(part 1 of 2)
# Autodesk Inventor assembly: FRC Fixed Field 2018_sldasm
Saved by Autodesk Inventor 2016 SP2 (Build 200236200, 236)
## iProperties
Created: 2018-01-13
Part Number: FRC Fixed Field 2018_sldasm
Document SubType Name: Assembly
Designer: CAD
Author: CAD
## Documents named in this file (943)
- C:\Users\CAD\Documents\GitHub\FIRST Power Up Field CAD\FRC Fixed Field 2018_sldasm.iam
- C:\Users\CAD\Documents\GitHub\FIRST Power Up Field CAD\Body_525_sldprt.ipt
- C:\Users\CAD\Documents\GitHub\FIRST Power Up Field CAD\Body_526_sldprt.ipt
- C:\Users\CAD\Documents\GitHub\FIRST Power Up Field CAD\Body_527_sldprt.ipt
- C:\Users\CAD\Documents\GitHub\FIRST Power Up Field CAD\Body_528_sldprt.ipt
- C:\Users\CAD\Documents\GitHub\FIRST Power Up Field CAD\Body_529_sldprt.ipt
- C:\Users\CAD\Documents\GitHub\FIRST Power Up Field CAD\Body_530_sldprt.ipt
- C:\Users\CAD\Documents\GitHub\FIRST Power Up Field CAD\Body_531_sldprt.ipt
- C:\Users\CAD\Documents\GitHub\FIRST Power Up Field CAD\Body_532_sldprt.ipt
- C:\Users\CAD\Documents\GitHub\FIRST Power Up Field CAD\Body_533_sldprt.ipt
- C:\Users\CAD\Documents\GitHub\FIRST Power Up Field CAD\Body_534_sldprt.ipt
- C:\Users\CAD\Documents\GitHub\FIRST Power Up Field CAD\Body_535_sldprt.ipt
- C:\Users\CAD\Documents\GitHub\FIRST Power Up Field CAD\Body_536_sldprt.ipt
- C:\Users\CAD\Documents\GitHub\FIRST Power Up Field CAD\Body_537_sldprt.ipt
- C:\Users\CAD\Documents\GitHub\FIRST Power Up Field CAD\Body_538_sldprt.ipt
- C:\Users\CAD\Documents\GitHub\FIRST Power Up Field CAD\Body_539_sldprt.ipt
- C:\Users\CAD\Documents\GitHub\FIRST Power Up Field CAD\Body_540_sldprt.ipt
- C:\Users\CAD\Documents\GitHub\FIRST Power Up Field CAD\Body_541_sldprt.ipt
- C:\Users\CAD\Documents\GitHub\FIRST Power Up Field CAD\Body_542_sldprt.ipt
- C:\Users\CAD\Documents\GitHub\FIRST Power Up Field CAD\Body_543_sldprt.ipt
- C:\Users\CAD\Documents\GitHub\FIRST Power Up Field CAD\Body_544_sldprt.ipt
- C:\Users\CAD\Documents\GitHub\FIRST Power Up Field CAD\Body_545_sldprt.ipt
- C:\Users\CAD\Documents\GitHub\FIRST Power Up Field CAD\Body_546_sldprt.ipt
- C:\Users\CAD\Documents\GitHub\FIRST Power Up Field CAD\Body_547_sldprt.ipt
- C:\Users\CAD\Documents\GitHub\FIRST Power Up Field CAD\Body_548_sldprt.ipt
- C:\Users\CAD\Documents\GitHub\FIRST Power Up Field CAD\Body_549_sldprt.ipt
- C:\Users\CAD\Documents\GitHub\FIRST Power Up Field CAD\Body_550_sldprt.ipt
- C:\Users\CAD\Documents\GitHub\FIRST Power Up Field CAD\Body_551_sldprt.ipt
- C:\Users\CAD\Documents\GitHub\FIRST Power Up Field CAD\Body_552_sldprt.ipt
- C:\Users\CAD\Documents\GitHub\FIRST Power Up Field CAD\Body_553_sldprt.ipt
- C:\Users\CAD\Documents\GitHub\FIRST Power Up Field CAD\Body_554_sldprt.ipt
- C:\Users\CAD\Documents\GitHub\FIRST Power Up Field CAD\Body_555_sldprt.ipt
- C:\Users\CAD\Documents\GitHub\FIRST Power Up Field CAD\Body_556_sldprt.ipt
- C:\Users\CAD\Documents\GitHub\FIRST Power Up Field CAD\Body_557_sldprt.ipt
- C:\Users\CAD\Documents\GitHub\FIRST Power Up Field CAD\Body_558_sldprt.ipt
- C:\Users\CAD\Documents\GitHub\FIRST Power Up Field CAD\Body_559_sldprt.ipt
- C:\Users\CAD\Documents\GitHub\FIRST Power Up Field CAD\Body_560_sldprt.ipt
- C:\Users\CAD\Documents\GitHub\FIRST Power Up Field CAD\Body_561_sldprt.ipt
- C:\Users\CAD\Documents\GitHub\FIRST Power Up Field CAD\Body_562_sldprt.ipt
- C:\Users\CAD\Documents\GitHub\FIRST Power Up Field CAD\Body_563_sldprt.ipt
- C:\Users\CAD\Documents\GitHub\FIRST Power Up Field CAD\Body_564_sldprt.ipt
- C:\Users\CAD\Documents\GitHub\FIRST Power Up Field CAD\Body_565_sldprt.ipt
- C:\Users\CAD\Documents\GitHub\FIRST Power Up Field CAD\Body_566_sldprt.ipt
- C:\Users\CAD\Documents\GitHub\FIRST Power Up Field CAD\Body_567_sldprt.ipt
- C:\Users\CAD\Documents\GitHub\FIRST Power Up Field CAD\Body_568_sldprt.ipt
- C:\Users\CAD\Documents\GitHub\FIRST Power Up Field CAD\Body_569_sldprt.ipt
- C:\Users\CAD\Documents\GitHub\FIRST Power Up Field CAD\Body_570_sldprt.ipt
- C:\Users\CAD\Documents\GitHub\FIRST Power Up Field CAD\Body_571_sldprt.ipt
- C:\Users\CAD\Documents\GitHub\FIRST Power Up Field CAD\Body_572_sldprt.ipt
- C:\Users\CAD\Documents\GitHub\FIRST Power Up Field CAD\Body_573_sldprt.ipt
- C:\Users\CAD\Documents\GitHub\FIRST Power Up Field CAD\Body_574_sldprt.ipt
- C:\Users\CAD\Documents\GitHub\FIRST Power Up Field CAD\Body_575_sldprt.ipt
- C:\Users\CAD\Documents\GitHub\FIRST Power Up Field CAD\Body_576_sldprt.ipt
- C:\Users\CAD\Documents\GitHub\FIRST Power Up Field CAD\Body_577_sldprt.ipt
- C:\Users\CAD\Documents\GitHub\FIRST Power Up Field CAD\Body_578_sldprt.ipt
- C:\Users\CAD\Documents\GitHub\FIRST Power Up Field CAD\Body_579_sldprt.ipt
- C:\Users\CAD\Documents\GitHub\FIRST Power Up Field CAD\Body_580_sldprt.ipt
- C:\Users\CAD\Documents\GitHub\FIRST Power Up Field CAD\Body_581_sldprt.ipt
- C:\Users\CAD\Documents\GitHub\FIRST Power Up Field CAD\Body_582_sldprt.ipt
- C:\Users\CAD\Documents\GitHub\FIRST Power Up Field CAD\Body_583_sldprt.ipt
- C:\Users\CAD\Documents\GitHub\FIRST Power Up Field CAD\Body_584_sldprt.ipt
- C:\Users\CAD\Documents\GitHub\FIRST Power Up Field CAD\Body_585_sldprt.ipt
- C:\Users\CAD\Documents\GitHub\FIRST Power Up Field CAD\Body_586_sldprt.ipt
- C:\Users\CAD\Documents\GitHub\FIRST Power Up Field CAD\Body_587_sldprt.ipt
- C:\Users\CAD\Documents\GitHub\FIRST Power Up Field CAD\Body_588_sldprt.ipt
- C:\Users\CAD\Documents\GitHub\FIRST Power Up Field CAD\Body_589_sldprt.ipt
- C:\Users\CAD\Documents\GitHub\FIRST Power Up Field CAD\Body_590_sldprt.ipt
- C:\Users\CAD\Documents\GitHub\FIRST Power Up Field CAD\Body_591_sldprt.ipt
- C:\Users\CAD\Documents\GitHub\FIRST Power Up Field CAD\Body_592_sldprt.ipt
- C:\Users\CAD\Documents\GitHub\FIRST Power Up Field CAD\Body_593_sldprt.ipt
- C:\Users\CAD\Documents\GitHub\FIRST Power Up Field CAD\Body_594_sldprt.ipt
- C:\Users\CAD\Documents\GitHub\FIRST Power Up Field CAD\Body_595_sldprt.ipt
- C:\Users\CAD\Documents\GitHub\FIRST Power Up Field CAD\Body_596_sldprt.ipt
- C:\Users\CAD\Documents\GitHub\FIRST Power Up Field CAD\Body_597_sldprt.ipt
- C:\Users\CAD\Documents\GitHub\FIRST Power Up Field CAD\Body_598_sldprt.ipt
- C:\Users\CAD\Documents\GitHub\FIRST Power Up Field CAD\Body_599_sldprt.ipt
- C:\Users\CAD\Documents\GitHub\FIRST Power Up Field CAD\Body_600_sldprt.ipt
- C:\Users\CAD\Documents\GitHub\FIRST Power Up Field CAD\Body_601_sldprt.ipt
- C:\Users\CAD\Documents\GitHub\FIRST Power Up Field CAD\Body_602_sldprt.ipt
- C:\Users\CAD\Documents\GitHub\FIRST Power Up Field CAD\Body_603_sldprt.ipt
- C:\Users\CAD\Documents\GitHub\FIRST Power Up Field CAD\Body_604_sldprt.ipt
- C:\Users\CAD\Documents\GitHub\FIRST Power Up Field CAD\Body_605_sldprt.ipt
- C:\Users\CAD\Documents\GitHub\FIRST Power Up Field CAD\Body_606_sldprt.ipt
- C:\Users\CAD\Documents\GitHub\FIRST Power Up Field CAD\Body_607_sldprt.ipt
- C:\Users\CAD\Documents\GitHub\FIRST Power Up Field CAD\Body_608_sldprt.ipt
- C:\Users\CAD\Documents\GitHub\FIRST Power Up Field CAD\Body_609_sldprt.ipt
- C:\Users\CAD\Documents\GitHub\FIRST Power Up Field CAD\Body_610_sldprt.ipt
- C:\Users\CAD\Documents\GitHub\FIRST Power Up Field CAD\Body_611_sldprt.ipt
- C:\Users\CAD\Documents\GitHub\FIRST Power Up Field CAD\Body_612_sldprt.ipt
- C:\Users\CAD\Documents\GitHub\FIRST Power Up Field CAD\Body_613_sldprt.ipt
- C:\Users\CAD\Documents\GitHub\FIRST Power Up Field CAD\Body_614_sldprt.ipt
- C:\Users\CAD\Documents\GitHub\FIRST Power Up Field CAD\Body_615_sldprt.ipt
- C:\Users\CAD\Documents\GitHub\FIRST Power Up Field CAD\Body_616_sldprt.ipt
- C:\Users\CAD\Documents\GitHub\FIRST Power Up Field CAD\Body_617_sldprt.ipt
- C:\Users\CAD\Documents\GitHub\FIRST Power Up Field CAD\Body_618_sldprt.ipt
- C:\Users\CAD\Documents\GitHub\FIRST Power Up Field CAD\Body_619_sldprt.ipt
- C:\Users\CAD\Documents\GitHub\FIRST Power Up Field CAD\Body_620_sldprt.ipt
- C:\Users\CAD\Documents\GitHub\FIRST Power Up Field CAD\Body_621_sldprt.ipt
- C:\Users\CAD\Documents\GitHub\FIRST Power Up Field CAD\Body_622_sldprt.ipt
- C:\Users\CAD\Documents\GitHub\FIRST Power Up Field CAD\Body_623_sldprt.ipt
- C:\Users\CAD\Documents\GitHub\FIRST Power Up Field CAD\Body_624_sldprt.ipt
- C:\Users\CAD\Documents\GitHub\FIRST Power Up Field CAD\Body_625_sldprt.ipt
- C:\Users\CAD\Documents\GitHub\FIRST Power Up Field CAD\Body_626_sldprt.ipt
- C:\Users\CAD\Documents\GitHub\FIRST Power Up Field CAD\Body_627_sldprt.ipt
- C:\Users\CAD\Documents\GitHub\FIRST Power Up Field CAD\Body_628_sldprt.ipt
- C:\Users\CAD\Documents\GitHub\FIRST Power Up Field CAD\Body_629_sldprt.ipt
- C:\Users\CAD\Documents\GitHub\FIRST Power Up Field CAD\Body_630_sldprt.ipt
- C:\Users\CAD\Documents\GitHub\FIRST Power Up Field CAD\Body_631_sldprt.ipt
- C:\Users\CAD\Documents\GitHub\FIRST Power Up Field CAD\Body_632_sldprt.ipt
- C:\Users\CAD\Documents\GitHub\FIRST Power Up Field CAD\Body_633_sldprt.ipt
- C:\Users\CAD\Documents\GitHub\FIRST Power Up Field CAD\Body_634_sldprt.ipt
- C:\Users\CAD\Documents\GitHub\FIRST Power Up Field CAD\Body_635_sldprt.ipt
- C:\Users\CAD\Documents\GitHub\FIRST Power Up Field CAD\Body_636_sldprt.ipt
- C:\Users\CAD\Documents\GitHub\FIRST Power Up Field CAD\Body_637_sldprt.ipt
- C:\Users\CAD\Documents\GitHub\FIRST Power Up Field CAD\Body_638_sldprt.ipt
- C:\Users\CAD\Documents\GitHub\FIRST Power Up Field CAD\Body_639_sldprt.ipt
- C:\Users\CAD\Documents\GitHub\FIRST Power Up Field CAD\Body_640_sldprt.ipt
- C:\Users\CAD\Documents\GitHub\FIRST Power Up Field CAD\Body_641_sldprt.ipt
- C:\Users\CAD\Documents\GitHub\FIRST Power Up Field CAD\Body_642_sldprt.ipt
- C:\Users\CAD\Documents\GitHub\FIRST Power Up Field CAD\Body_643_sldprt.ipt
- C:\Users\CAD\Documents\GitHub\FIRST Power Up Field CAD\Body_644_sldprt.ipt
- C:\Users\CAD\Documents\GitHub\FIRST Power Up Field CAD\Body_645_sldprt.ipt
- C:\Users\CAD\Documents\GitHub\FIRST Power Up Field CAD\Body_646_sldprt.ipt
- C:\Users\CAD\Documents\GitHub\FIRST Power Up Field CAD\Body_647_sldprt.ipt
- C:\Users\CAD\Documents\GitHub\FIRST Power Up Field CAD\Body_648_sldprt.ipt
- C:\Users\CAD\Documents\GitHub\FIRST Power Up Field CAD\Body_649_sldprt.ipt
- C:\Users\CAD\Documents\GitHub\FIRST Power Up Field CAD\Body_650_sldprt.ipt
- C:\Users\CAD\Documents\GitHub\FIRST Power Up Field CAD\Body_651_sldprt.ipt
- C:\Users\CAD\Documents\GitHub\FIRST Power Up Field CAD\Body_652_sldprt.ipt
- C:\Users\CAD\Documents\GitHub\FIRST Power Up Field CAD\Body_653_sldprt.ipt
- C:\Users\CAD\Documents\GitHub\FIRST Power Up Field CAD\Body_654_sldprt.ipt
- C:\Users\CAD\Documents\GitHub\FIRST Power Up Field CAD\Body_655_sldprt.ipt
- C:\Users\CAD\Documents\GitHub\FIRST Power Up Field CAD\Body_656_sldprt.ipt
- C:\Users\CAD\Documents\GitHub\FIRST Power Up Field CAD\Body_657_sldprt.ipt
- C:\Users\CAD\Documents\GitHub\FIRST Power Up Field CAD\Body_658_sldprt.ipt
- C:\Users\CAD\Documents\GitHub\FIRST Power Up Field CAD\Body_659_sldprt.ipt
- C:\Users\CAD\Documents\GitHub\FIRST Power Up Field CAD\Body_660_sldprt.ipt
- C:\Users\CAD\Documents\GitHub\FIRST Power Up Field CAD\Body_661_sldprt.ipt
- C:\Users\CAD\Documents\GitHub\FIRST Power Up Field CAD\Body_662_sldprt.ipt
- C:\Users\CAD\Documents\GitHub\FIRST Power Up Field CAD\Body_663_sldprt.ipt
- C:\Users\CAD\Documents\GitHub\FIRST Power Up Field CAD\Body_664_sldprt.ipt
- C:\Users\CAD\Documents\GitHub\FIRST Power Up Field CAD\Body_665_sldprt.ipt
- C:\Users\CAD\Documents\GitHub\FIRST Power Up Field CAD\Body_666_sldprt.ipt
- C:\Users\CAD\Documents\GitHub\FIRST Power Up Field CAD\Body_667_sldprt.ipt
- C:\Users\CAD\Documents\GitHub\FIRST Power Up Field CAD\Body_668_sldprt.ipt
- C:\Users\CAD\Documents\GitHub\FIRST Power Up Field CAD\Body_669_sldprt.ipt
- C:\Users\CAD\Documents\GitHub\FIRST Power Up Field CAD\Body_670_sldprt.ipt
- C:\Users\CAD\Documents\GitHub\FIRST Power Up Field CAD\Body_671_sldprt.ipt
- C:\Users\CAD\Documents\GitHub\FIRST Power Up Field CAD\Body_672_sldprt.ipt
- C:\Users\CAD\Documents\GitHub\FIRST Power Up Field CAD\Body_673_sldprt.ipt
- C:\Users\CAD\Documents\GitHub\FIRST Power Up Field CAD\Body_674_sldprt.ipt
- C:\Users\CAD\Documents\GitHub\FIRST Power Up Field CAD\Body_675_sldprt.ipt
- C:\Users\CAD\Documents\GitHub\FIRST Power Up Field CAD\Body_676_sldprt.ipt
- C:\Users\CAD\Documents\GitHub\FIRST Power Up Field CAD\Body_677_sldprt.ipt
- C:\Users\CAD\Documents\GitHub\FIRST Power Up Field CAD\Body_678_sldprt.ipt
- C:\Users\CAD\Documents\GitHub\FIRST Power Up Field CAD\Body_679_sldprt.ipt
- C:\Users\CAD\Documents\GitHub\FIRST Power Up Field CAD\Body_680_sldprt.ipt
- C:\Users\CAD\Documents\GitHub\FIRST Power Up Field CAD\Body_681_sldprt.ipt
- C:\Users\CAD\Documents\GitHub\FIRST Power Up Field CAD\Body_682_sldprt.ipt
- C:\Users\CAD\Documents\GitHub\FIRST Power Up Field CAD\Body_683_sldprt.ipt
- C:\Users\CAD\Documents\GitHub\FIRST Power Up Field CAD\Body_684_sldprt.ipt
- C:\Users\CAD\Documents\GitHub\FIRST Power Up Field CAD\Body_685_sldprt.ipt
- C:\Users\CAD\Documents\GitHub\FIRST Power Up Field CAD\Body_686_sldprt.ipt
- C:\Users\CAD\Documents\GitHub\FIRST Power Up Field CAD\Body_687_sldprt.ipt
- C:\Users\CAD\Documents\GitHub\FIRST Power Up Field CAD\Body_688_sldprt.ipt
- C:\Users\CAD\Documents\GitHub\FIRST Power Up Field CAD\Body_689_sldprt.ipt
- C:\Users\CAD\Documents\GitHub\FIRST Power Up Field CAD\Body_690_sldprt.ipt
- C:\Users\CAD\Documents\GitHub\FIRST Power Up Field CAD\Body_691_sldprt.ipt
- C:\Users\CAD\Documents\GitHub\FIRST Power Up Field CAD\Body_692_sldprt.ipt
- C:\Users\CAD\Documents\GitHub\FIRST Power Up Field CAD\Body_693_sldprt.ipt
- C:\Users\CAD\Documents\GitHub\FIRST Power Up Field CAD\Body_694_sldprt.ipt
- C:\Users\CAD\Documents\GitHub\FIRST Power Up Field CAD\Body_695_sldprt.ipt
- C:\Users\CAD\Documents\GitHub\FIRST Power Up Field CAD\Body_696_sldprt.ipt
- C:\Users\CAD\Documents\GitHub\FIRST Power Up Field CAD\Body_697_sldprt.ipt
- C:\Users\CAD\Documents\GitHub\FIRST Power Up Field CAD\Body_698_sldprt.ipt
- C:\Users\CAD\Documents\GitHub\FIRST Power Up Field CAD\Body_699_sldprt.ipt
- C:\Users\CAD\Documents\GitHub\FIRST Power Up Field CAD\Body_700_sldprt.ipt
- C:\Users\CAD\Documents\GitHub\FIRST Power Up Field CAD\Body_701_sldprt.ipt
- C:\Users\CAD\Documents\GitHub\FIRST Power Up Field CAD\Body_702_sldprt.ipt
- C:\Users\CAD\Documents\GitHub\FIRST Power Up Field CAD\Body_703_sldprt.ipt
- C:\Users\CAD\Documents\GitHub\FIRST Power Up Field CAD\Body_704_sldprt.ipt
- C:\Users\CAD\Documents\GitHub\FIRST Power Up Field CAD\Body_705_sldprt.ipt
- C:\Users\CAD\Documents\GitHub\FIRST Power Up Field CAD\Body_706_sldprt.ipt
- C:\Users\CAD\Documents\GitHub\FIRST Power Up Field CAD\Body_707_sldprt.ipt
- C:\Users\CAD\Documents\GitHub\FIRST Power Up Field CAD\Body_708_sldprt.ipt
- C:\Users\CAD\Documents\GitHub\FIRST Power Up Field CAD\Body_709_sldprt.ipt
- C:\Users\CAD\Documents\GitHub\FIRST Power Up Field CAD\Body_710_sldprt.ipt
- C:\Users\CAD\Documents\GitHub\FIRST Power Up Field CAD\Body_711_sldprt.ipt
- C:\Users\CAD\Documents\GitHub\FIRST Power Up Field CAD\Body_712_sldprt.ipt
- C:\Users\CAD\Documents\GitHub\FIRST Power Up Field CAD\Body_713_sldprt.ipt
- C:\Users\CAD\Documents\GitHub\FIRST Power Up Field CAD\Body_714_sldprt.ipt
- C:\Users\CAD\Documents\GitHub\FIRST Power Up Field CAD\Body_715_sldprt.ipt
- C:\Users\CAD\Documents\GitHub\FIRST Power Up Field CAD\Body_716_sldprt.ipt
- C:\Users\CAD\Documents\GitHub\FIRST Power Up Field CAD\Body_717_sldprt.ipt
- C:\Users\CAD\Documents\GitHub\FIRST Power Up Field CAD\Body_718_sldprt.ipt
- C:\Users\CAD\Documents\GitHub\FIRST Power Up Field CAD\Body_719_sldprt.ipt
- C:\Users\CAD\Documents\GitHub\FIRST Power Up Field CAD\Body_720_sldprt.ipt
- C:\Users\CAD\Documents\GitHub\FIRST Power Up Field CAD\Body_721_sldprt.ipt
- C:\Users\CAD\Documents\GitHub\FIRST Power Up Field CAD\Body_722_sldprt.ipt
- C:\Users\CAD\Documents\GitHub\FIRST Power Up Field CAD\Body_723_sldprt.ipt
- C:\Users\CAD\Documents\GitHub\FIRST Power Up Field CAD\Body_724_sldprt.ipt
- C:\Users\CAD\Documents\GitHub\FIRST Power Up Field CAD\Body_725_sldprt.ipt
- C:\Users\CAD\Documents\GitHub\FIRST Power Up Field CAD\Body_726_sldprt.ipt
- C:\Users\CAD\Documents\GitHub\FIRST Power Up Field CAD\Body_727_sldprt.ipt
- C:\Users\CAD\Documents\GitHub\FIRST Power Up Field CAD\Body_728_sldprt.ipt
- C:\Users\CAD\Documents\GitHub\FIRST Power Up Field CAD\Body_729_sldprt.ipt
- C:\Users\CAD\Documents\GitHub\FIRST Power Up Field CAD\Body_730_sldprt.ipt
- C:\Users\CAD\Documents\GitHub\FIRST Power Up Field CAD\Body_731_sldprt.ipt
- C:\Users\CAD\Documents\GitHub\FIRST Power Up Field CAD\Body_732_sldprt.ipt
- C:\Users\CAD\Documents\GitHub\FIRST Power Up Field CAD\Body_733_sldprt.ipt
- C:\Users\CAD\Documents\GitHub\FIRST Power Up Field CAD\Body_734_sldprt.ipt
- C:\Users\CAD\Documents\GitHub\FIRST Power Up Field CAD\Body_735_sldprt.ipt
- C:\Users\CAD\Documents\GitHub\FIRST Power Up Field CAD\Body_736_sldprt.ipt
- C:\Users\CAD\Documents\GitHub\FIRST Power Up Field CAD\Body_737_sldprt.ipt
- C:\Users\CAD\Documents\GitHub\FIRST Power Up Field CAD\Body_738_sldprt.ipt
- C:\Users\CAD\Documents\GitHub\FIRST Power Up Field CAD\Body_739_sldprt.ipt
- C:\Users\CAD\Documents\GitHub\FIRST Power Up Field CAD\Body_740_sldprt.ipt
- C:\Users\CAD\Documents\GitHub\FIRST Power Up Field CAD\Body_741_sldprt.ipt
- C:\Users\CAD\Documents\GitHub\FIRST Power Up Field CAD\Body_742_sldprt.ipt
- C:\Users\CAD\Documents\GitHub\FIRST Power Up Field CAD\Body_743_sldprt.ipt
- C:\Users\CAD\Documents\GitHub\FIRST Power Up Field CAD\Body_744_sldprt.ipt
- C:\Users\CAD\Documents\GitHub\FIRST Power Up Field CAD\Body_745_sldprt.ipt
- C:\Users\CAD\Documents\GitHub\FIRST Power Up Field CAD\Body_746_sldprt.ipt
- C:\Users\CAD\Documents\GitHub\FIRST Power Up Field CAD\Body_747_sldprt.ipt
- C:\Users\CAD\Documents\GitHub\FIRST Power Up Field CAD\Body_748_sldprt.ipt
- C:\Users\CAD\Documents\GitHub\FIRST Power Up Field CAD\Body_749_sldprt.ipt
- C:\Users\CAD\Documents\GitHub\FIRST Power Up Field CAD\Body_750_sldprt.ipt
- C:\Users\CAD\Documents\GitHub\FIRST Power Up Field CAD\Body_751_sldprt.ipt
- C:\Users\CAD\Documents\GitHub\FIRST Power Up Field CAD\Body_752_sldprt.ipt
- C:\Users\CAD\Documents\GitHub\FIRST Power Up Field CAD\Body_753_sldprt.ipt
- C:\Users\CAD\Documents\GitHub\FIRST Power Up Field CAD\Body_754_sldprt.ipt
- C:\Users\CAD\Documents\GitHub\FIRST Power Up Field CAD\Body_755_sldprt.ipt
- C:\Users\CAD\Documents\GitHub\FIRST Power Up Field CAD\Body_756_sldprt.ipt
- C:\Users\CAD\Documents\GitHub\FIRST Power Up Field CAD\Body_757_sldprt.ipt
- C:\Users\CAD\Documents\GitHub\FIRST Power Up Field CAD\Body_758_sldprt.ipt
- C:\Users\CAD\Documents\GitHub\FIRST Power Up Field CAD\Body_759_sldprt.ipt
- C:\Users\CAD\Documents\GitHub\FIRST Power Up Field CAD\Body_760_sldprt.ipt
- C:\Users\CAD\Documents\GitHub\FIRST Power Up Field CAD\Body_761_sldprt.ipt
- C:\Users\CAD\Documents\GitHub\FIRST Power Up Field CAD\Body_762_sldprt.ipt
- C:\Users\CAD\Documents\GitHub\FIRST Power Up Field CAD\Body_763_sldprt.ipt
- C:\Users\CAD\Documents\GitHub\FIRST Power Up Field CAD\Body_764_sldprt.ipt
- C:\Users\CAD\Documents\GitHub\FIRST Power Up Field CAD\Body_765_sldprt.ipt
- C:\Users\CAD\Documents\GitHub\FIRST Power Up Field CAD\Body_766_sldprt.ipt
- C:\Users\CAD\Documents\GitHub\FIRST Power Up Field CAD\Body_767_sldprt.ipt
- C:\Users\CAD\Documents\GitHub\FIRST Power Up Field CAD\Body_768_sldprt.ipt
- C:\Users\CAD\Documents\GitHub\FIRST Power Up Field CAD\Body_769_sldprt.ipt
- C:\Users\CAD\Documents\GitHub\FIRST Power Up Field CAD\Body_770_sldprt.ipt
- C:\Users\CAD\Documents\GitHub\FIRST Power Up Field CAD\Body_771_sldprt.ipt
- C:\Users\CAD\Documents\GitHub\FIRST Power Up Field CAD\Body_772_sldprt.ipt
- C:\Users\CAD\Documents\GitHub\FIRST Power Up Field CAD\Body_773_sldprt.ipt
- C:\Users\CAD\Documents\GitHub\FIRST Power Up Field CAD\Body_774_sldprt.ipt
- C:\Users\CAD\Documents\GitHub\FIRST Power Up Field CAD\Body_775_sldprt.ipt
- C:\Users\CAD\Documents\GitHub\FIRST Power Up Field CAD\Body_776_sldprt.ipt
- C:\Users\CAD\Documents\GitHub\FIRST Power Up Field CAD\Body_777_sldprt.ipt
- C:\Users\CAD\Documents\GitHub\FIRST Power Up Field CAD\Body_778_sldprt.ipt
- C:\Users\CAD\Documents\GitHub\FIRST Power Up Field CAD\Body_779_sldprt.ipt
- C:\Users\CAD\Documents\GitHub\FIRST Power Up Field CAD\Body_780_sldprt.ipt
- C:\Users\CAD\Documents\GitHub\FIRST Power Up Field CAD\Body_781_sldprt.ipt
- C:\Users\CAD\Documents\GitHub\FIRST Power Up Field CAD\Body_782_sldprt.ipt
- C:\Users\CAD\Documents\GitHub\FIRST Power Up Field CAD\Body_783_sldprt.ipt
- C:\Users\CAD\Documents\GitHub\FIRST Power Up Field CAD\Body_784_sldprt.ipt
- C:\Users\CAD\Documents\GitHub\FIRST Power Up Field CAD\Body_785_sldprt.ipt
- C:\Users\CAD\Documents\GitHub\FIRST Power Up Field CAD\Body_786_sldprt.ipt
- C:\Users\CAD\Documents\GitHub\FIRST Power Up Field CAD\Body_787_sldprt.ipt
- C:\Users\CAD\Documents\GitHub\FIRST Power Up Field CAD\Body_788_sldprt.ipt
- C:\Users\CAD\Documents\GitHub\FIRST Power Up Field CAD\Body_789_sldprt.ipt
- C:\Users\CAD\Documents\GitHub\FIRST Power Up Field CAD\Body_790_sldprt.ipt
- C:\Users\CAD\Documents\GitHub\FIRST Power Up Field CAD\Body_791_sldprt.ipt
- C:\Users\CAD\Documents\GitHub\FIRST Power Up Field CAD\Body_792_sldprt.ipt
- C:\Users\CAD\Documents\GitHub\FIRST Power Up Field CAD\Body_793_sldprt.ipt
- C:\Users\CAD\Documents\GitHub\FIRST Power Up Field CAD\Body_794_sldprt.ipt
- C:\Users\CAD\Documents\GitHub\FIRST Power Up Field CAD\Body_795_sldprt.ipt
- C:\Users\CAD\Documents\GitHub\FIRST Power Up Field CAD\Body_796_sldprt.ipt
- C:\Users\CAD\Documents\GitHub\FIRST Power Up Field CAD\Body_797_sldprt.ipt
- C:\Users\CAD\Documents\GitHub\FIRST Power Up Field CAD\Body_798_sldprt.ipt
- C:\Users\CAD\Documents\GitHub\FIRST Power Up Field CAD\Body_799_sldprt.ipt
- C:\Users\CAD\Documents\GitHub\FIRST Power Up Field CAD\Body_800_sldprt.ipt
- C:\Users\CAD\Documents\GitHub\FIRST Power Up Field CAD\Body_801_sldprt.ipt
- C:\Users\CAD\Documents\GitHub\FIRST Power Up Field CAD\Body_802_sldprt.ipt
- C:\Users\CAD\Documents\GitHub\FIRST Power Up Field CAD\Body_803_sldprt.ipt
- C:\Users\CAD\Documents\GitHub\FIRST Power Up Field CAD\Body_804_sldprt.ipt
- C:\Users\CAD\Documents\GitHub\FIRST Power Up Field CAD\Body_805_sldprt.ipt
- C:\Users\CAD\Documents\GitHub\FIRST Power Up Field CAD\Body_806_sldprt.ipt
- C:\Users\CAD\Documents\GitHub\FIRST Power Up Field CAD\Body_807_sldprt.ipt
- C:\Users\CAD\Documents\GitHub\FIRST Power Up Field CAD\Body_808_sldprt.ipt
- C:\Users\CAD\Documents\GitHub\FIRST Power Up Field CAD\Body_809_sldprt.ipt
- C:\Users\CAD\Documents\GitHub\FIRST Power Up Field CAD\Body_810_sldprt.ipt
- C:\Users\CAD\Documents\GitHub\FIRST Power Up Field CAD\Body_811_sldprt.ipt
- C:\Users\CAD\Documents\GitHub\FIRST Power Up Field CAD\Body_812_sldprt.ipt
- C:\Users\CAD\Documents\GitHub\FIRST Power Up Field CAD\Body_813_sldprt.ipt
- C:\Users\CAD\Documents\GitHub\FIRST Power Up Field CAD\Body_814_sldprt.ipt
- C:\Users\CAD\Documents\GitHub\FIRST Power Up Field CAD\Body_815_sldprt.ipt
- C:\Users\CAD\Documents\GitHub\FIRST Power Up Field CAD\Body_816_sldprt.ipt
- C:\Users\CAD\Documents\GitHub\FIRST Power Up Field CAD\Body_817_sldprt.ipt
- C:\Users\CAD\Documents\GitHub\FIRST Power Up Field CAD\Body_818_sldprt.ipt
- C:\Users\CAD\Documents\GitHub\FIRST Power Up Field CAD\Body_819_sldprt.ipt
- C:\Users\CAD\Documents\GitHub\FIRST Power Up Field CAD\Body_820_sldprt.ipt
- C:\Users\CAD\Documents\GitHub\FIRST Power Up Field CAD\Body_821_sldprt.ipt
- C:\Users\CAD\Documents\GitHub\FIRST Power Up Field CAD\Body_822_sldprt.ipt
- C:\Users\CAD\Documents\GitHub\FIRST Power Up Field CAD\Body_823_sldprt.ipt
- C:\Users\CAD\Documents\GitHub\FIRST Power Up Field CAD\Body_824_sldprt.ipt
- C:\Users\CAD\Documents\GitHub\FIRST Power Up Field CAD\Body_825_sldprt.ipt
- C:\Users\CAD\Documents\GitHub\FIRST Power Up Field CAD\Body_826_sldprt.ipt
- C:\Users\CAD\Documents\GitHub\FIRST Power Up Field CAD\Body_827_sldprt.ipt
- C:\Users\CAD\Documents\GitHub\FIRST Power Up Field CAD\Body_828_sldprt.ipt
- C:\Users\CAD\Documents\GitHub\FIRST Power Up Field CAD\Body_829_sldprt.ipt
- C:\Users\CAD\Documents\GitHub\FIRST Power Up Field CAD\Body_830_sldprt.ipt
- C:\Users\CAD\Documents\GitHub\FIRST Power Up Field CAD\Body_831_sldprt.ipt
- C:\Users\CAD\Documents\GitHub\FIRST Power Up Field CAD\Body_832_sldprt.ipt
- C:\Users\CAD\Documents\GitHub\FIRST Power Up Field CAD\Body_833_sldprt.ipt
- C:\Users\CAD\Documents\GitHub\FIRST Power Up Field CAD\Body_834_sldprt.ipt
- C:\Users\CAD\Documents\GitHub\FIRST Power Up Field CAD\Body_835_sldprt.ipt
- C:\Users\CAD\Documents\GitHub\FIRST Power Up Field CAD\Body_836_sldprt.ipt
- C:\Users\CAD\Documents\GitHub\FIRST Power Up Field CAD\Body_837_sldprt.ipt
- C:\Users\CAD\Documents\GitHub\FIRST Power Up Field CAD\Body_838_sldprt.ipt
- C:\Users\CAD\Documents\GitHub\FIRST Power Up Field CAD\Body_839_sldprt.ipt
- C:\Users\CAD\Documents\GitHub\FIRST Power Up Field CAD\Body_840_sldprt.ipt
- C:\Users\CAD\Documents\GitHub\FIRST Power Up Field CAD\Body_841_sldprt.ipt
- C:\Users\CAD\Documents\GitHub\FIRST Power Up Field CAD\Body_842_sldprt.ipt
- C:\Users\CAD\Documents\GitHub\FIRST Power Up Field CAD\Body_843_sldprt.ipt
- C:\Users\CAD\Documents\GitHub\FIRST Power Up Field CAD\Body_844_sldprt.ipt
- C:\Users\CAD\Documents\GitHub\FIRST Power Up Field CAD\Body_845_sldprt.ipt
- C:\Users\CAD\Documents\GitHub\FIRST Power Up Field CAD\Body_846_sldprt.ipt
- C:\Users\CAD\Documents\GitHub\FIRST Power Up Field CAD\Body_847_sldprt.ipt
- C:\Users\CAD\Documents\GitHub\FIRST Power Up Field CAD\Body_848_sldprt.ipt
- C:\Users\CAD\Documents\GitHub\FIRST Power Up Field CAD\Body_849_sldprt.ipt
- C:\Users\CAD\Documents\GitHub\FIRST Power Up Field CAD\Body_850_sldprt.ipt
- C:\Users\CAD\Documents\GitHub\FIRST Power Up Field CAD\Body_851_sldprt.ipt
- C:\Users\CAD\Documents\GitHub\FIRST Power Up Field CAD\Body_852_sldprt.ipt
- C:\Users\CAD\Documents\GitHub\FIRST Power Up Field CAD\Body_853_sldprt.ipt
- C:\Users\CAD\Documents\GitHub\FIRST Power Up Field CAD\Body_854_sldprt.ipt
- C:\Users\CAD\Documents\GitHub\FIRST Power Up Field CAD\Body_855_sldprt.ipt
- C:\Users\CAD\Documents\GitHub\FIRST Power Up Field CAD\Body_856_sldprt.ipt
- C:\Users\CAD\Documents\GitHub\FIRST Power Up Field CAD\Body_857_sldprt.ipt
- C:\Users\CAD\Documents\GitHub\FIRST Power Up Field CAD\Body_858_sldprt.ipt
- C:\Users\CAD\Documents\GitHub\FIRST Power Up Field CAD\Body_859_sldprt.ipt
- C:\Users\CAD\Documents\GitHub\FIRST Power Up Field CAD\Body_860_sldprt.ipt
- C:\Users\CAD\Documents\GitHub\FIRST Power Up Field CAD\Body_861_sldprt.ipt
- C:\Users\CAD\Documents\GitHub\FIRST Power Up Field CAD\Body_862_sldprt.ipt
- C:\Users\CAD\Documents\GitHub\FIRST Power Up Field CAD\Body_863_sldprt.ipt
- C:\Users\CAD\Documents\GitHub\FIRST Power Up Field CAD\Body_864_sldprt.ipt
- C:\Users\CAD\Documents\GitHub\FIRST Power Up Field CAD\Body_865_sldprt.ipt
- C:\Users\CAD\Documents\GitHub\FIRST Power Up Field CAD\Body_866_sldprt.ipt
- C:\Users\CAD\Documents\GitHub\FIRST Power Up Field CAD\Body_867_sldprt.ipt
- C:\Users\CAD\Documents\GitHub\FIRST Power Up Field CAD\Body_868_sldprt.ipt
- C:\Users\CAD\Documents\GitHub\FIRST Power Up Field CAD\Body_869_sldprt.ipt
- C:\Users\CAD\Documents\GitHub\FIRST Power Up Field CAD\Body_870_sldprt.ipt
- C:\Users\CAD\Documents\GitHub\FIRST Power Up Field CAD\Body_871_sldprt.ipt
- C:\Users\CAD\Documents\GitHub\FIRST Power Up Field CAD\Body_872_sldprt.ipt
- C:\Users\CAD\Documents\GitHub\FIRST Power Up Field CAD\Body_873_sldprt.ipt
- C:\Users\CAD\Documents\GitHub\FIRST Power Up Field CAD\Body_874_sldprt.ipt
- C:\Users\CAD\Documents\GitHub\FIRST Power Up Field CAD\Body_875_sldprt.ipt
- C:\Users\CAD\Documents\GitHub\FIRST Power Up Field CAD\Body_876_sldprt.ipt
- C:\Users\CAD\Documents\GitHub\FIRST Power Up Field CAD\Body_877_sldprt.ipt
- C:\Users\CAD\Documents\GitHub\FIRST Power Up Field CAD\Body_878_sldprt.ipt
- C:\Users\CAD\Documents\GitHub\FIRST Power Up Field CAD\Body_879_sldprt.ipt
- C:\Users\CAD\Documents\GitHub\FIRST Power Up Field CAD\Body_880_sldprt.ipt
- C:\Users\CAD\Documents\GitHub\FIRST Power Up Field CAD\Body_881_sldprt.ipt
- C:\Users\CAD\Documents\GitHub\FIRST Power Up Field CAD\Body_882_sldprt.ipt
- C:\Users\CAD\Documents\GitHub\FIRST Power Up Field CAD\Body_883_sldprt.ipt
- C:\Users\CAD\Documents\GitHub\FIRST Power Up Field CAD\Body_884_sldprt.ipt
- C:\Users\CAD\Documents\GitHub\FIRST Power Up Field CAD\Body_885_sldprt.ipt
- C:\Users\CAD\Documents\GitHub\FIRST Power Up Field CAD\Body_886_sldprt.ipt
- C:\Users\CAD\Documents\GitHub\FIRST Power Up Field CAD\Body_887_sldprt.ipt
- C:\Users\CAD\Documents\GitHub\FIRST Power Up Field CAD\Body_888_sldprt.ipt
- C:\Users\CAD\Documents\GitHub\FIRST Power Up Field CAD\Body_889_sldprt.ipt
- C:\Users\CAD\Documents\GitHub\FIRST Power Up Field CAD\Body_890_sldprt.ipt
- C:\Users\CAD\Documents\GitHub\FIRST Power Up Field CAD\Body_891_sldprt.ipt
- C:\Users\CAD\Documents\GitHub\FIRST Power Up Field CAD\Body_892_sldprt.ipt
- C:\Users\CAD\Documents\GitHub\FIRST Power Up Field CAD\Body_893_sldprt.ipt
- C:\Users\CAD\Documents\GitHub\FIRST Power Up Field CAD\Body_894_sldprt.ipt
- C:\Users\CAD\Documents\GitHub\FIRST Power Up Field CAD\Body_895_sldprt.ipt
- C:\Users\CAD\Documents\GitHub\FIRST Power Up Field CAD\Body_896_sldprt.ipt
- C:\Users\CAD\Documents\GitHub\FIRST Power Up Field CAD\Body_897_sldprt.ipt
- C:\Users\CAD\Documents\GitHub\FIRST Power Up Field CAD\Body_898_sldprt.ipt
- C:\Users\CAD\Documents\GitHub\FIRST Power Up Field CAD\Body_899_sldprt.ipt
- C:\Users\CAD\Documents\GitHub\FIRST Power Up Field CAD\Body_900_sldprt.ipt
- C:\Users\CAD\Documents\GitHub\FIRST Power Up Field CAD\Body_901_sldprt.ipt
- C:\Users\CAD\Documents\GitHub\FIRST Power Up Field CAD\Body_902_sldprt.ipt
- C:\Users\CAD\Documents\GitHub\FIRST Power Up Field CAD\Body_903_sldprt.ipt
- C:\Users\CAD\Documents\GitHub\FIRST Power Up Field CAD\Body_904_sldprt.ipt
- C:\Users\CAD\Documents\GitHub\FIRST Power Up Field CAD\Body_905_sldprt.ipt
- C:\Users\CAD\Documents\GitHub\FIRST Power Up Field CAD\Body_906_sldprt.ipt
- C:\Users\CAD\Documents\GitHub\FIRST Power Up Field CAD\Body_907_sldprt.ipt
- C:\Users\CAD\Documents\GitHub\FIRST Power Up Field CAD\Body_908_sldprt.ipt
- C:\Users\CAD\Documents\GitHub\FIRST Power Up Field CAD\Body_909_sldprt.ipt
- C:\Users\CAD\Documents\GitHub\FIRST Power Up Field CAD\Body_910_sldprt.ipt
- C:\Users\CAD\Documents\GitHub\FIRST Power Up Field CAD\Body_911_sldprt.ipt
- C:\Users\CAD\Documents\GitHub\FIRST Power Up Field CAD\Body_912_sldprt.ipt
- C:\Users\CAD\Documents\GitHub\FIRST Power Up Field CAD\Body_913_sldprt.ipt
- C:\Users\CAD\Documents\GitHub\FIRST Power Up Field CAD\Body_914_sldprt.ipt
- C:\Users\CAD\Documents\GitHub\FIRST Power Up Field CAD\Body_915_sldprt.ipt
- C:\Users\CAD\Documents\GitHub\FIRST Power Up Field CAD\Body_916_sldprt.ipt
- C:\Users\CAD\Documents\GitHub\FIRST Power Up Field CAD\Body_917_sldprt.ipt
- C:\Users\CAD\Documents\GitHub\FIRST Power Up Field CAD\Body_918_sldprt.ipt
- C:\Users\CAD\Documents\GitHub\FIRST Power Up Field CAD\Body_919_sldprt.ipt
- C:\Users\CAD\Documents\GitHub\FIRST Power Up Field CAD\Body_920_sldprt.ipt
- C:\Users\CAD\Documents\GitHub\FIRST Power Up Field CAD\Body_921_sldprt.ipt
- C:\Users\CAD\Documents\GitHub\FIRST Power Up Field CAD\Body_922_sldprt.ipt
- C:\Users\CAD\Documents\GitHub\FIRST Power Up Field CAD\Body_923_sldprt.ipt
- C:\Users\CAD\Documents\GitHub\FIRST Power Up Field CAD\Body_924_sldprt.ipt
- C:\Users\CAD\Documents\GitHub\FIRST Power Up Field CAD\Body_925_sldprt.ipt
- C:\Users\CAD\Documents\GitHub\FIRST Power Up Field CAD\Body_926_sldprt.ipt
- C:\Users\CAD\Documents\GitHub\FIRST Power Up Field CAD\Body_927_sldprt.ipt
- C:\Users\CAD\Documents\GitHub\FIRST Power Up Field CAD\Body_928_sldprt.ipt
- C:\Users\CAD\Documents\GitHub\FIRST Power Up Field CAD\Body_929_sldprt.ipt
- C:\Users\CAD\Documents\GitHub\FIRST Power Up Field CAD\Body_930_sldprt.ipt
- C:\Users\CAD\Documents\GitHub\FIRST Power Up Field CAD\Body_931_sldprt.ipt
- C:\Users\CAD\Documents\GitHub\FIRST Power Up Field CAD\Body_932_sldprt.ipt
- C:\Users\CAD\Documents\GitHub\FIRST Power Up Field CAD\Body_933_sldprt.ipt
- C:\Users\CAD\Documents\GitHub\FIRST Power Up Field CAD\Body_934_sldprt.ipt
- C:\Users\CAD\Documents\GitHub\FIRST Power Up Field CAD\Body_935_sldprt.ipt
- C:\Users\CAD\Documents\GitHub\FIRST Power Up Field CAD\Body_936_sldprt.ipt
- C:\Users\CAD\Documents\GitHub\FIRST Power Up Field CAD\Body_937_sldprt.ipt
- C:\Users\CAD\Documents\GitHub\FIRST Power Up Field CAD\Body_938_sldprt.ipt
- C:\Users\CAD\Documents\GitHub\FIRST Power Up Field CAD\Body_939_sldprt.ipt
- C:\Users\CAD\Documents\GitHub\FIRST Power Up Field CAD\Body_940_sldprt.ipt
- C:\Users\CAD\Documents\GitHub\FIRST Power Up Field CAD\Body_941_sldprt.ipt
- C:\Users\CAD\Documents\GitHub\FIRST Power Up Field CAD\Body_942_sldprt.ipt
- C:\Users\CAD\Documents\GitHub\FIRST Power Up Field CAD\Body_943_sldprt.ipt
- C:\Users\CAD\Documents\GitHub\FIRST Power Up Field CAD\Body_944_sldprt.ipt
- C:\Users\CAD\Documents\GitHub\FIRST Power Up Field CAD\Body_945_sldprt.ipt
- C:\Users\CAD\Documents\GitHub\FIRST Power Up Field CAD\Body_946_sldprt.ipt
- C:\Users\CAD\Documents\GitHub\FIRST Power Up Field CAD\Body_947_sldprt.ipt
- C:\Users\CAD\Documents\GitHub\FIRST Power Up Field CAD\Body_948_sldprt.ipt
- C:\Users\CAD\Documents\GitHub\FIRST Power Up Field CAD\Body_949_sldprt.ipt
- C:\Users\CAD\Documents\GitHub\FIRST Power Up Field CAD\Body_950_sldprt.ipt
- C:\Users\CAD\Documents\GitHub\FIRST Power Up Field CAD\Body_951_sldprt.ipt
- C:\Users\CAD\Documents\GitHub\FIRST Power Up Field CAD\Body_952_sldprt.ipt
- C:\Users\CAD\Documents\GitHub\FIRST Power Up Field CAD\Body_953_sldprt.ipt
- C:\Users\CAD\Documents\GitHub\FIRST Power Up Field CAD\Body_954_sldprt.ipt
- C:\Users\CAD\Documents\GitHub\FIRST Power Up Field CAD\Body_955_sldprt.ipt
- C:\Users\CAD\Documents\GitHub\FIRST Power Up Field CAD\Body_956_sldprt.ipt
- C:\Users\CAD\Documents\GitHub\FIRST Power Up Field CAD\Body_957_sldprt.ipt
- C:\Users\CAD\Documents\GitHub\FIRST Power Up Field CAD\Body_958_sldprt.ipt
- C:\Users\CAD\Documents\GitHub\FIRST Power Up Field CAD\Body_959_sldprt.ipt
- C:\Users\CAD\Documents\GitHub\FIRST Power Up Field CAD\Body_960_sldprt.ipt
- C:\Users\CAD\Documents\GitHub\FIRST Power Up Field CAD\Body_961_sldprt.ipt
- C:\Users\CAD\Documents\GitHub\FIRST Power Up Field CAD\Body_962_sldprt.ipt
- C:\Users\CAD\Documents\GitHub\FIRST Power Up Field CAD\Body_963_sldprt.ipt
- C:\Users\CAD\Documents\GitHub\FIRST Power Up Field CAD\Body_964_sldprt.ipt
- C:\Users\CAD\Documents\GitHub\FIRST Power Up Field CAD\Body_965_sldprt.ipt
- C:\Users\CAD\Documents\GitHub\FIRST Power Up Field CAD\Body_966_sldprt.ipt
- C:\Users\CAD\Documents\GitHub\FIRST Power Up Field CAD\Body_967_sldprt.ipt
- C:\Users\CAD\Documents\GitHub\FIRST Power Up Field CAD\Body_968_sldprt.ipt
- C:\Users\CAD\Documents\GitHub\FIRST Power Up Field CAD\Body_969_sldprt.ipt
- C:\Users\CAD\Documents\GitHub\FIRST Power Up Field CAD\Body_970_sldprt.ipt
- C:\Users\CAD\Documents\GitHub\FIRST Power Up Field CAD\Body_971_sldprt.ipt
- C:\Users\CAD\Documents\GitHub\FIRST Power Up Field CAD\Body_972_sldprt.ipt
- C:\Users\CAD\Documents\GitHub\FIRST Power Up Field CAD\Body_973_sldprt.ipt
- C:\Users\CAD\Documents\GitHub\FIRST Power Up Field CAD\Body_974_sldprt.ipt
- C:\Users\CAD\Documents\GitHub\FIRST Power Up Field CAD\Body_975_sldprt.ipt
- C:\Users\CAD\Documents\GitHub\FIRST Power Up Field CAD\Body_976_sldprt.ipt
- C:\Users\CAD\Documents\GitHub\FIRST Power Up Field CAD\Body_977_sldprt.ipt
- C:\Users\CAD\Documents\GitHub\FIRST Power Up Field CAD\Body_978_sldprt.ipt
- C:\Users\CAD\Documents\GitHub\FIRST Power Up Field CAD\Body_979_sldprt.ipt
- C:\Users\CAD\Documents\GitHub\FIRST Power Up Field CAD\Body_980_sldprt.ipt
- C:\Users\CAD\Documents\GitHub\FIRST Power Up Field CAD\Body_981_sldprt.ipt
- C:\Users\CAD\Documents\GitHub\FIRST Power Up Field CAD\Body_982_sldprt.ipt
- C:\Users\CAD\Documents\GitHub\FIRST Power Up Field CAD\Body_983_sldprt.ipt
- C:\Users\CAD\Documents\GitHub\FIRST Power Up Field CAD\Body_984_sldprt.ipt
- C:\Users\CAD\Documents\GitHub\FIRST Power Up Field CAD\Body_985_sldprt.ipt
- C:\Users\CAD\Documents\GitHub\FIRST Power Up Field CAD\Body_986_sldprt.ipt
- C:\Users\CAD\Documents\GitHub\FIRST Power Up Field CAD\Body_987_sldprt.ipt
- C:\Users\CAD\Documents\GitHub\FIRST Power Up Field CAD\Body_988_sldprt.ipt
- C:\Users\CAD\Documents\GitHub\FIRST Power Up Field CAD\Body_989_sldprt.ipt
- C:\Users\CAD\Documents\GitHub\FIRST Power Up Field CAD\Body_990_sldprt.ipt
- C:\Users\CAD\Documents\GitHub\FIRST Power Up Field CAD\Body_991_sldprt.ipt
- C:\Users\CAD\Documents\GitHub\FIRST Power Up Field CAD\Body_992_sldprt.ipt
- C:\Users\CAD\Documents\GitHub\FIRST Power Up Field CAD\Body_993_sldprt.ipt
- C:\Users\CAD\Documents\GitHub\FIRST Power Up Field CAD\Body_994_sldprt.ipt
- C:\Users\CAD\Documents\GitHub\FIRST Power Up Field CAD\Body_995_sldprt.ipt
- C:\Users\CAD\Documents\GitHub\FIRST Power Up Field CAD\Body_996_sldprt.ipt
- C:\Users\CAD\Documents\GitHub\FIRST Power Up Field CAD\Body_997_sldprt.ipt
- C:\Users\CAD\Documents\GitHub\FIRST Power Up Field CAD\Body_998_sldprt.ipt
- C:\Users\CAD\Documents\GitHub\FIRST Power Up Field CAD\Body_999_sldprt.ipt
- C:\Users\CAD\Documents\GitHub\FIRST Power Up Field CAD\Body_1000_sldprt.ipt
- C:\Users\CAD\Documents\GitHub\FIRST Power Up Field CAD\Body_1001_sldprt.ipt
- C:\Users\CAD\Documents\GitHub\FIRST Power Up Field CAD\Body_1002_sldprt.ipt
- C:\Users\CAD\Documents\GitHub\FIRST Power Up Field CAD\Body_1003_sldprt.ipt
- C:\Users\CAD\Documents\GitHub\FIRST Power Up Field CAD\Body_1004_sldprt.ipt
- C:\Users\CAD\Documents\GitHub\FIRST Power Up Field CAD\Body_1005_sldprt.ipt
- C:\Users\CAD\Documents\GitHub\FIRST Power Up Field CAD\Body_1006_sldprt.ipt
- C:\Users\CAD\Documents\GitHub\FIRST Power Up Field CAD\Body_1007_sldprt.ipt
- C:\Users\CAD\Documents\GitHub\FIRST Power Up Field CAD\Body_1008_sldprt.ipt
- C:\Users\CAD\Documents\GitHub\FIRST Power Up Field CAD\Body_1009_sldprt.ipt
- C:\Users\CAD\Documents\GitHub\FIRST Power Up Field CAD\Body_1010_sldprt.ipt
- C:\Users\CAD\Documents\GitHub\FIRST Power Up Field CAD\Body_1011_sldprt.ipt
- C:\Users\CAD\Documents\GitHub\FIRST Power Up Field CAD\Body_1012_sldprt.ipt
- C:\Users\CAD\Documents\GitHub\FIRST Power Up Field CAD\Body_1013_sldprt.ipt
- C:\Users\CAD\Documents\GitHub\FIRST Power Up Field CAD\Body_1014_sldprt.ipt
- C:\Users\CAD\Documents\GitHub\FIRST Power Up Field CAD\Body_1015_sldprt.ipt
- C:\Users\CAD\Documents\GitHub\FIRST Power Up Field CAD\Body_1016_sldprt.ipt
- C:\Users\CAD\Documents\GitHub\FIRST Power Up Field CAD\Body_1017_sldprt.ipt
- C:\Users\CAD\Documents\GitHub\FIRST Power Up Field CAD\Body_1018_sldprt.ipt
- C:\Users\CAD\Documents\GitHub\FIRST Power Up Field CAD\Body_1019_sldprt.ipt
- C:\Users\CAD\Documents\GitHub\FIRST Power Up Field CAD\Body_1020_sldprt.ipt
- C:\Users\CAD\Documents\GitHub\FIRST Power Up Field CAD\Body_1021_sldprt.ipt
- C:\Users\CAD\Documents\GitHub\FIRST Power Up Field CAD\Body_1022_sldprt.ipt
- C:\Users\CAD\Documents\GitHub\FIRST Power Up Field CAD\Body_1023_sldprt.ipt
- C:\Users\CAD\Documents\GitHub\FIRST Power Up Field CAD\Body_1024_sldprt.ipt
- C:\Users\CAD\Documents\GitHub\FIRST Power Up Field CAD\Body_1025_sldprt.ipt
- C:\Users\CAD\Documents\GitHub\FIRST Power Up Field CAD\Body_1026_sldprt.ipt
- C:\Users\CAD\Documents\GitHub\FIRST Power Up Field CAD\Body_1027_sldprt.ipt
- C:\Users\CAD\Documents\GitHub\FIRST Power Up Field CAD\Body_1028_sldprt.ipt
- C:\Users\CAD\Documents\GitHub\FIRST Power Up Field CAD\Body_1029_sldprt.ipt
- C:\Users\CAD\Documents\GitHub\FIRST Power Up Field CAD\Body_1030_sldprt.ipt
- C:\Users\CAD\Documents\GitHub\FIRST Power Up Field CAD\Body_1031_sldprt.ipt
- C:\Users\CAD\Documents\GitHub\FIRST Power Up Field CAD\Body_1032_sldprt.ipt
- C:\Users\CAD\Documents\GitHub\FIRST Power Up Field CAD\Body_1033_sldprt.ipt
- C:\Users\CAD\Documents\GitHub\FIRST Power Up Field CAD\Body_1034_sldprt.ipt
- C:\Users\CAD\Documents\GitHub\FIRST Power Up Field CAD\Body_1035_sldprt.ipt
- C:\Users\CAD\Documents\GitHub\FIRST Power Up Field CAD\Body_1036_sldprt.ipt
- C:\Users\CAD\Documents\GitHub\FIRST Power Up Field CAD\Body_1037_sldprt.ipt
- C:\Users\CAD\Documents\GitHub\FIRST Power Up Field CAD\Body_1038_sldprt.ipt
- C:\Users\CAD\Documents\GitHub\FIRST Power Up Field CAD\Body_1039_sldprt.ipt
- C:\Users\CAD\Documents\GitHub\FIRST Power Up Field CAD\Body_1040_sldprt.ipt
- C:\Users\CAD\Documents\GitHub\FIRST Power Up Field CAD\Body_1041_sldprt.ipt
- C:\Users\CAD\Documents\GitHub\FIRST Power Up Field CAD\Body_1042_sldprt.ipt
- C:\Users\CAD\Documents\GitHub\FIRST Power Up Field CAD\Body_1043_sldprt.ipt
- C:\Users\CAD\Documents\GitHub\FIRST Power Up Field CAD\Body_1044_sldprt.ipt
- C:\Users\CAD\Documents\GitHub\FIRST Power Up Field CAD\Body_1045_sldprt.ipt
- C:\Users\CAD\Documents\GitHub\FIRST Power Up Field CAD\Body_1046_sldprt.ipt
- C:\Users\CAD\Documents\GitHub\FIRST Power Up Field CAD\Body_1047_sldprt.ipt
- C:\Users\CAD\Documents\GitHub\FIRST Power Up Field CAD\Body_1048_sldprt.ipt
- C:\Users\CAD\Documents\GitHub\FIRST Power Up Field CAD\Body_1049_sldprt.ipt
- C:\Users\CAD\Documents\GitHub\FIRST Power Up Field CAD\Body_1050_sldprt.ipt
- C:\Users\CAD\Documents\GitHub\FIRST Power Up Field CAD\Body_1051_sldprt.ipt
- C:\Users\CAD\Documents\GitHub\FIRST Power Up Field CAD\Body_1052_sldprt.ipt
- C:\Users\CAD\Documents\GitHub\FIRST Power Up Field CAD\Body_1053_sldprt.ipt
- C:\Users\CAD\Documents\GitHub\FIRST Power Up Field CAD\Body_1054_sldprt.ipt
- C:\Users\CAD\Documents\GitHub\FIRST Power Up Field CAD\Body_1055_sldprt.ipt
- C:\Users\CAD\Documents\GitHub\FIRST Power Up Field CAD\Body_1056_sldprt.ipt
- C:\Users\CAD\Documents\GitHub\FIRST Power Up Field CAD\Body_1057_sldprt.ipt
- C:\Users\CAD\Documents\GitHub\FIRST Power Up Field CAD\Body_1058_sldprt.ipt
- C:\Users\CAD\Documents\GitHub\FIRST Power Up Field CAD\Body_1059_sldprt.ipt
- C:\Users\CAD\Documents\GitHub\FIRST Power Up Field CAD\Body_1060_sldprt.ipt
- C:\Users\CAD\Documents\GitHub\FIRST Power Up Field CAD\Body_1061_sldprt.ipt
- C:\Users\CAD\Documents\GitHub\FIRST Power Up Field CAD\Body_1062_sldprt.ipt
- C:\Users\CAD\Documents\GitHub\FIRST Power Up Field CAD\Body_1063_sldprt.ipt
- C:\Users\CAD\Documents\GitHub\FIRST Power Up Field CAD\Body_1064_sldprt.ipt
- C:\Users\CAD\Documents\GitHub\FIRST Power Up Field CAD\Body_1065_sldprt.ipt
- C:\Users\CAD\Documents\GitHub\FIRST Power Up Field CAD\Body_1066_sldprt.ipt
- C:\Users\CAD\Documents\GitHub\FIRST Power Up Field CAD\Body_1067_sldprt.ipt
- C:\Users\CAD\Documents\GitHub\FIRST Power Up Field CAD\Body_1068_sldprt.ipt
- C:\Users\CAD\Documents\GitHub\FIRST Power Up Field CAD\Body_1069_sldprt.ipt
- C:\Users\CAD\Documents\GitHub\FIRST Power Up Field CAD\Body_1070_sldprt.ipt
- C:\Users\CAD\Documents\GitHub\FIRST Power Up Field CAD\Body_1071_sldprt.ipt
- C:\Users\CAD\Documents\GitHub\FIRST Power Up Field CAD\Body_1072_sldprt.ipt
- C:\Users\CAD\Documents\GitHub\FIRST Power Up Field CAD\Body_1073_sldprt.ipt
- C:\Users\CAD\Documents\GitHub\FIRST Power Up Field CAD\Body_1074_sldprt.ipt
- C:\Users\CAD\Documents\GitHub\FIRST Power Up Field CAD\Body_1075_sldprt.ipt
- C:\Users\CAD\Documents\GitHub\FIRST Power Up Field CAD\Body_1076_sldprt.ipt
- C:\Users\CAD\Documents\GitHub\FIRST Power Up Field CAD\Body_1077_sldprt.ipt
- C:\Users\CAD\Documents\GitHub\FIRST Power Up Field CAD\Body_1078_sldprt.ipt
- C:\Users\CAD\Documents\GitHub\FIRST Power Up Field CAD\Body_1079_sldprt.ipt
- C:\Users\CAD\Documents\GitHub\FIRST Power Up Field CAD\Body_1080_sldprt.ipt
- C:\Users\CAD\Documents\GitHub\FIRST Power Up Field CAD\Body_1081_sldprt.ipt
- C:\Users\CAD\Documents\GitHub\FIRST Power Up Field CAD\Body_1082_sldprt.ipt
- C:\Users\CAD\Documents\GitHub\FIRST Power Up Field CAD\Body_1083_sldprt.ipt
- C:\Users\CAD\Documents\GitHub\FIRST Power Up Field CAD\Body_1084_sldprt.ipt
- C:\Users\CAD\Documents\GitHub\FIRST Power Up Field CAD\Body_1085_sldprt.ipt
- C:\Users\CAD\Documents\GitHub\FIRST Power Up Field CAD\Body_1086_sldprt.ipt
- C:\Users\CAD\Documents\GitHub\FIRST Power Up Field CAD\Body_1087_sldprt.ipt
- C:\Users\CAD\Documents\GitHub\FIRST Power Up Field CAD\Body_1088_sldprt.ipt
- C:\Users\CAD\Documents\GitHub\FIRST Power Up Field CAD\Body_1089_sldprt.ipt
- C:\Users\CAD\Documents\GitHub\FIRST Power Up Field CAD\Body_1090_sldprt.ipt
- C:\Users\CAD\Documents\GitHub\FIRST Power Up Field CAD\Body_1091_sldprt.ipt
- C:\Users\CAD\Documents\GitHub\FIRST Power Up Field CAD\Body_1092_sldprt.ipt
- C:\Users\CAD\Documents\GitHub\FIRST Power Up Field CAD\Body_1093_sldprt.ipt
- C:\Users\CAD\Documents\GitHub\FIRST Power Up Field CAD\Body_1094_sldprt.ipt
- C:\Users\CAD\Documents\GitHub\FIRST Power Up Field CAD\Body_1095_sldprt.ipt
- C:\Users\CAD\Documents\GitHub\FIRST Power Up Field CAD\Body_1096_sldprt.ipt
- C:\Users\CAD\Documents\GitHub\FIRST Power Up Field CAD\Body_1097_sldprt.ipt
- C:\Users\CAD\Documents\GitHub\FIRST Power Up Field CAD\Body_1098_sldprt.ipt
- C:\Users\CAD\Documents\GitHub\FIRST Power Up Field CAD\Body_1099_sldprt.ipt
- C:\Users\CAD\Documents\GitHub\FIRST Power Up Field CAD\Body_1100_sldprt.ipt
- C:\Users\CAD\Documents\GitHub\FIRST Power Up Field CAD\Body_1101_sldprt.ipt
- C:\Users\CAD\Documents\GitHub\FIRST Power Up Field CAD\Body_1102_sldprt.ipt
- C:\Users\CAD\Documents\GitHub\FIRST Power Up Field CAD\Body_1103_sldprt.ipt
- C:\Users\CAD\Documents\GitHub\FIRST Power Up Field CAD\Body_1104_sldprt.ipt
- C:\Users\CAD\Documents\GitHub\FIRST Power Up Field CAD\Body_1105_sldprt.ipt
- C:\Users\CAD\Documents\GitHub\FIRST Power Up Field CAD\Body_1106_sldprt.ipt
- C:\Users\CAD\Documents\GitHub\FIRST Power Up Field CAD\Body_1107_sldprt.ipt
- C:\Users\CAD\Documents\GitHub\FIRST Power Up Field CAD\Body_1108_sldprt.ipt
- C:\Users\CAD\Documents\GitHub\FIRST Power Up Field CAD\Body_1109_sldprt.ipt
- C:\Users\CAD\Documents\GitHub\FIRST Power Up Field CAD\Body_1110_sldprt.ipt
- C:\Users\CAD\Documents\GitHub\FIRST Power Up Field CAD\Body_1111_sldprt.ipt
- C:\Users\CAD\Documents\GitHub\FIRST Power Up Field CAD\Body_1112_sldprt.ipt
- C:\Users\CAD\Documents\GitHub\FIRST Power Up Field CAD\Body_1113_sldprt.ipt
- C:\Users\CAD\Documents\GitHub\FIRST Power Up Field CAD\Body_1114_sldprt.ipt
- C:\Users\CAD\Documents\GitHub\FIRST Power Up Field CAD\Body_1115_sldprt.ipt
- C:\Users\CAD\Documents\GitHub\FIRST Power Up Field CAD\Body_1116_sldprt.ipt
- C:\Users\CAD\Documents\GitHub\FIRST Power Up Field CAD\Body_1117_sldprt.ipt
- C:\Users\CAD\Documents\GitHub\FIRST Power Up Field CAD\Body_1118_sldprt.ipt
- C:\Users\CAD\Documents\GitHub\FIRST Power Up Field CAD\Body_1119_sldprt.ipt
- C:\Users\CAD\Documents\GitHub\FIRST Power Up Field CAD\Body_1120_sldprt.ipt
- C:\Users\CAD\Documents\GitHub\FIRST Power Up Field CAD\Body_1121_sldprt.ipt
- C:\Users\CAD\Documents\GitHub\FIRST Power Up Field CAD\Body_1122_sldprt.ipt
- C:\Users\CAD\Documents\GitHub\FIRST Power Up Field CAD\Body_1123_sldprt.ipt
- C:\Users\CAD\Documents\GitHub\FIRST Power Up Field CAD\Body_1124_sldprt.ipt
- C:\Users\CAD\Documents\GitHub\FIRST Power Up Field CAD\Body_1125_sldprt.ipt
- C:\Users\CAD\Documents\GitHub\FIRST Power Up Field CAD\Body_1126_sldprt.ipt
- C:\Users\CAD\Documents\GitHub\FIRST Power Up Field CAD\Body_1127_sldprt.ipt
- C:\Users\CAD\Documents\GitHub\FIRST Power Up Field CAD\Body_1128_sldprt.ipt
- C:\Users\CAD\Documents\GitHub\FIRST Power Up Field CAD\Body_1129_sldprt.ipt
- C:\Users\CAD\Documents\GitHub\FIRST Power Up Field CAD\Body_1130_sldprt.ipt
- C:\Users\CAD\Documents\GitHub\FIRST Power Up Field CAD\Body_1131_sldprt.ipt
- C:\Users\CAD\Documents\GitHub\FIRST Power Up Field CAD\Body_1132_sldprt.ipt
- C:\Users\CAD\Documents\GitHub\FIRST Power Up Field CAD\Body_1133_sldprt.ipt
- C:\Users\CAD\Documents\GitHub\FIRST Power Up Field CAD\Body_1134_sldprt.ipt
- C:\Users\CAD\Documents\GitHub\FIRST Power Up Field CAD\Body_1135_sldprt.ipt
- C:\Users\CAD\Documents\GitHub\FIRST Power Up Field CAD\Body_1136_sldprt.ipt
- C:\Users\CAD\Documents\GitHub\FIRST Power Up Field CAD\Body_1137_sldprt.ipt
- C:\Users\CAD\Documents\GitHub\FIRST Power Up Field CAD\Body_1138_sldprt.ipt
- C:\Users\CAD\Documents\GitHub\FIRST Power Up Field CAD\Body_1139_sldprt.ipt
- C:\Users\CAD\Documents\GitHub\FIRST Power Up Field CAD\Body_1140_sldprt.ipt
- C:\Users\CAD\Documents\GitHub\FIRST Power Up Field CAD\Body_1141_sldprt.ipt
- C:\Users\CAD\Documents\GitHub\FIRST Power Up Field CAD\Body_1142_sldprt.ipt
- C:\Users\CAD\Documents\GitHub\FIRST Power Up Field CAD\Body_1143_sldprt.ipt
- C:\Users\CAD\Documents\GitHub\FIRST Power Up Field CAD\Body_1144_sldprt.ipt
- C:\Users\CAD\Documents\GitHub\FIRST Power Up Field CAD\Body_1145_sldprt.ipt
- C:\Users\CAD\Documents\GitHub\FIRST Power Up Field CAD\Body_1146_sldprt.ipt
- C:\Users\CAD\Documents\GitHub\FIRST Power Up Field CAD\Body_1147_sldprt.ipt
- C:\Users\CAD\Documents\GitHub\FIRST Power Up Field CAD\Body_1148_sldprt.ipt
- C:\Users\CAD\Documents\GitHub\FIRST Power Up Field CAD\Body_1149_sldprt.ipt
- C:\Users\CAD\Documents\GitHub\FIRST Power Up Field CAD\Body_1150_sldprt.ipt
- C:\Users\CAD\Documents\GitHub\FIRST Power Up Field CAD\Body_1151_sldprt.ipt
- C:\Users\CAD\Documents\GitHub\FIRST Power Up Field CAD\Body_1152_sldprt.ipt
- C:\Users\CAD\Documents\GitHub\FIRST Power Up Field CAD\Body_1153_sldprt.ipt
- C:\Users\CAD\Documents\GitHub\FIRST Power Up Field CAD\Body_1154_sldprt.ipt
- C:\Users\CAD\Documents\GitHub\FIRST Power Up Field CAD\Body_1155_sldprt.ipt
- C:\Users\CAD\Documents\GitHub\FIRST Power Up Field CAD\Body_1156_sldprt.ipt
- C:\Users\CAD\Documents\GitHub\FIRST Power Up Field CAD\Body_1157_sldprt.ipt
- C:\Users\CAD\Documents\GitHub\FIRST Power Up Field CAD\Body_1158_sldprt.ipt
- C:\Users\CAD\Documents\GitHub\FIRST Power Up Field CAD\Body_1159_sldprt.ipt
- C:\Users\CAD\Documents\GitHub\FIRST Power Up Field CAD\Body_1160_sldprt.ipt
- C:\Users\CAD\Documents\GitHub\FIRST Power Up Field CAD\Body_1161_sldprt.ipt
- C:\Users\CAD\Documents\GitHub\FIRST Power Up Field CAD\Body_1162_sldprt.ipt
- C:\Users\CAD\Documents\GitHub\FIRST Power Up Field CAD\Body_1163_sldprt.ipt
- C:\Users\CAD\Documents\GitHub\FIRST Power Up Field CAD\Body_1164_sldprt.ipt